# Autodesk Inventor assembly: Battery Pack
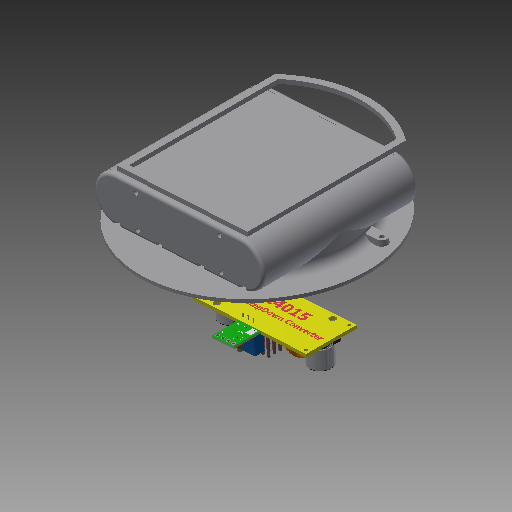
[picture p0: Inventor's stored thumbnail of the model, 512x512]
Saved by Autodesk Inventor 2018 (Build 220112000, 112)
## iProperties
Created: 2017-08-21
Part Number: Battery Pack
Material: Generisch
Document SubType Name: Assembly
Designer: JochenAlt
Author: JochenAlt
## Documents named in this file (5)
- D:\Projects\Manfred\design\cad\Inventor\Battery Pack.iam
- D:\Projects\Manfred\design\cad\Inventor\Battery 18650.ipt
- D:\Projects\Manfred\design\cad\Inventor\BatterPackHolder.ipt
- D:\Projects\Manfred\design\cad\Inventor\XL4015 DC-DC StepDown Assembly.iam
- D:\Projects\Manfred\design\cad\Inventor\Pololu 2843 5V Step Down Regulator.ipt
## Components (7 placed, 4 different names)
1. Battery 18650:1 — Passend:2, Fluchtend:5, Fluchtend:6
2. Battery 18650:2 — Passend:1, Fluchtend:5, Fluchtend:8, Fluchtend:9
3. Battery 18650:3 — Passend:3, Fluchtend:6, Fluchtend:7
4. Battery 18650:4 — Passend:4, Fluchtend:7
5. BatterPackHolder:1 — Fluchtend:4, Passend:1, Passend:2, Passend:3, Passend:4, Fluchtend:8, Passend:5, Passend:6, Winkel:1, Passend:7, Fluchtend:9, Passend:9
6. XL4015 DC-DC StepDown Assembly:1 [sub-assembly] — Passend:5, Passend:6, Winkel:1, Passend:8, Passend:9
7. Pololu 2843 5V Step Down Regulator:1 — Passend:7, Passend:8
## Relationships (16: Mate 9, Flush 6, Angle 1)
- Fluchtend:4 [Flush]: BatterPackHolder:1
- Passend:1 [Mate]: Battery 18650:2 ↔ BatterPackHolder:1
- Passend:2 [Mate]: Battery 18650:1 ↔ BatterPackHolder:1
- Passend:3 [Mate]: Battery 18650:3 ↔ BatterPackHolder:1
- Passend:4 [Mate]: Battery 18650:4 ↔ BatterPackHolder:1
- Fluchtend:5 [Flush]: Battery 18650:1 ↔ Battery 18650:2
- Fluchtend:6 [Flush]: Battery 18650:1 ↔ Battery 18650:3
- Fluchtend:7 [Flush]: Battery 18650:3 ↔ Battery 18650:4
- Fluchtend:8 [Flush] (1 mm): Battery 18650:2 ↔ BatterPackHolder:1
- Passend:5 [Mate]: BatterPackHolder:1 ↔ XL4015 DC-DC StepDown Assembly:1
- Passend:6 [Mate]: BatterPackHolder:1 ↔ XL4015 DC-DC StepDown Assembly:1
- Winkel:1 [Angle] (0 deg): BatterPackHolder:1 ↔ XL4015 DC-DC StepDown Assembly:1
- Passend:7 [Mate]: BatterPackHolder:1 ↔ Pololu 2843 5V Step Down Regulator:1
- Passend:8 [Mate]: XL4015 DC-DC StepDown Assembly:1 ↔ Pololu 2843 5V Step Down Regulator:1
- Fluchtend:9 [Flush]: Battery 18650:2 ↔ BatterPackHolder:1
- Passend:9 [Mate]: BatterPackHolder:1 ↔ XL4015 DC-DC StepDown Assembly:1
